# Autodesk Inventor assembly: Versaframe 26x30
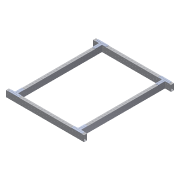
[picture p0: Inventor's stored thumbnail of the model, 180x180]
Saved by Autodesk Inventor 2015 (Build 190159000, 159)
## iProperties
Created: 2014-12-02
Part Number: Versaframe 26x30
Document SubType Name: Assembly
Designer: Nemo
Author: Nemo
## Documents named in this file (4)
- H:\Nemo\Documents\Robotics\CAD Files\Tutorial Folder\Versaframe 26x30.iam
- H:\Nemo\Documents\Robotics\CAD Files\Tutorial Folder\VersaFrame practice side rail 28 in.ipt
- H:\Nemo\Documents\Robotics\CAD Files\Tutorial Folder\VersaFrame practice end rail 26 in.ipt
- H:\Nemo\Documents\Robotics\CAD Files\Tutorial Folder\COTS Parts\VersaFrame\VersaFrame Tee Gusset.ipt
## Components (8 placed, 5 different names)
1. Right - VersaFrame practice side rail 28 in:1 — Flush:1, Flush:2, Mate:1, Symmetry:1, Flush:3, Flush:5, Flush:6, Mate:2
2. Left - VersaFrame practice side rail 28 in:2 — Flush:2, Mate:1, Symmetry:1
3. Front - VersaFrame practice end rail 26 in:1 — Flush:4, Flush:5, Flush:6, Mate:2, Flush:7, Mate:3, Symmetry:2, Insert:3, Mate:6, Insert:4, Mate:7
4. Back - VersaFrame practice end rail 26 in:2 — Flush:7, Mate:3, Symmetry:2, Insert:1, Mate:4, Insert:2, Mate:5
5. VersaFrame Tee Gusset:1 — Insert:1, Mate:4
6. VersaFrame Tee Gusset:2 — Insert:2, Mate:5
7. VersaFrame Tee Gusset:3 — Insert:3, Mate:6
8. VersaFrame Tee Gusset:4 — Insert:4, Mate:7
## Relationships (20: Flush 7, Mate 7, Insert 4, Symmetry 2)
- Flush:1 (50.8 mm): Right - VersaFrame practice side rail 28 in:1
- Flush:2: Right - VersaFrame practice side rail 28 in:1 ↔ Left - VersaFrame practice side rail 28 in:2
- Mate:1: Right - VersaFrame practice side rail 28 in:1 ↔ Left - VersaFrame practice side rail 28 in:2
- Symmetry:1: Right - VersaFrame practice side rail 28 in:1 ↔ Left - VersaFrame practice side rail 28 in:2
- Flush:3: Right - VersaFrame practice side rail 28 in:1
- Flush:4: Front - VersaFrame practice end rail 26 in:1
- Flush:5: Right - VersaFrame practice side rail 28 in:1 ↔ Front - VersaFrame practice end rail 26 in:1
- Flush:6 (50.8 mm): Right - VersaFrame practice side rail 28 in:1 ↔ Front - VersaFrame practice end rail 26 in:1
- Mate:2: Right - VersaFrame practice side rail 28 in:1 ↔ Front - VersaFrame practice end rail 26 in:1
- Flush:7: Front - VersaFrame practice end rail 26 in:1 ↔ Back - VersaFrame practice end rail 26 in:2
- Mate:3: Front - VersaFrame practice end rail 26 in:1 ↔ Back - VersaFrame practice end rail 26 in:2
- Symmetry:2: Front - VersaFrame practice end rail 26 in:1 ↔ Back - VersaFrame practice end rail 26 in:2
- Insert:1: Back - VersaFrame practice end rail 26 in:2 ↔ VersaFrame Tee Gusset:1
- Mate:4: Back - VersaFrame practice end rail 26 in:2 ↔ VersaFrame Tee Gusset:1
- Insert:2: Back - VersaFrame practice end rail 26 in:2 ↔ VersaFrame Tee Gusset:2
- Mate:5: Back - VersaFrame practice end rail 26 in:2 ↔ VersaFrame Tee Gusset:2
- Insert:3: Front - VersaFrame practice end rail 26 in:1 ↔ VersaFrame Tee Gusset:3
- Mate:6: Front - VersaFrame practice end rail 26 in:1 ↔ VersaFrame Tee Gusset:3
- Insert:4: Front - VersaFrame practice end rail 26 in:1 ↔ VersaFrame Tee Gusset:4
- Mate:7: Front - VersaFrame practice end rail 26 in:1 ↔ VersaFrame Tee Gusset:4
